# Autodesk Inventor assembly: Full_Field_V5.3_Full_Detail
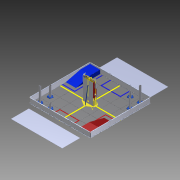
[picture p0: Inventor's stored thumbnail of the model, 180x180]
Saved by Autodesk Inventor 2015 (Build 190159000, 159)
## iProperties
Created: 2015-04-21
Part Number: Full_Field_V5.3_Full_Detail
Document SubType Name: Assembly
Designer: David Tenney
Author: David Tenney
Title: LR15 Full Field V5.3 Full Detail.STEP
Description: STEP AP214
Creation Date: 2014-09-08
Sending System: SolidWorks 2014
Preprocessor: SwSTEP 2.0
## Documents named in this file (10)
- C:\Users\David Tenney\Documents\GitHub\CAD\Field\Imported Components\Full_Field_V5.3_Full_Detail\Full_Field_V5.3_Full_Detail.iam
- C:\Users\David Tenney\Documents\GitHub\CAD\Field\Imported Components\Full_Field_V5.3_Full_Detail\Center Tower 4.4r.iam
- C:\Users\David Tenney\Documents\GitHub\CAD\Field\Imported Components\Full_Field_V5.3_Full_Detail\Bucket ramp v4.iam
- C:\Users\David Tenney\Documents\GitHub\CAD\Field\Imported Components\Full_Field_V5.3_Full_Detail\Player Station.ipt
- C:\Users\David Tenney\Documents\GitHub\CAD\Field\Imported Components\Full_Field_V5.3_Full_Detail\Final Rev1 - Pentagon Goal - 30cm.iam
- C:\Users\David Tenney\Documents\GitHub\CAD\Field\Imported Components\Full_Field_V5.3_Full_Detail\Final Rev1 - Pentagon Goal - 90cm.iam
- C:\Users\David Tenney\Documents\GitHub\CAD\Field\Imported Components\Full_Field_V5.3_Full_Detail\Final Rev1 - Pentagon Goal - 60cm.iam
- C:\Users\David Tenney\Documents\GitHub\CAD\Field\Imported Components\Full_Field_V5.3_Full_Detail\FTC Field Asm.iam
- C:\Users\David Tenney\Documents\GitHub\CAD\Field\Tile Field.iam
- C:\Users\David Tenney\Documents\GitHub\CAD\Field\Bucket ramp v4 Blue.iam
## Components (13 placed, 13 different names)
1. Tile Field_1 [sub-assembly] — Mate:5, Mate:6, Mate:7, Mate:8, Mate:9, Mate:10
2. Center Tower 4.4r_2 [sub-assembly] — Mate:10, Angle:1, Mate:11
3. Bucket ramp v4_3 [sub-assembly] — Mate:3, Mate:4, Mate:6
4. Bucket ramp v4_4 [sub-assembly] — Mate:1, Mate:2, Mate:5
5. Player Station_5
6. Player Station_6
7. Final Rev1 - Pentagon Goal - 30cm_7 [sub-assembly]
8. Final Rev1 - Pentagon Goal - 90cm_8 [sub-assembly]
9. Final Rev1 - Pentagon Goal - 60cm_9 [sub-assembly]
10. Final Rev1 - Pentagon Goal - 30cm_10 [sub-assembly]
11. Final Rev1 - Pentagon Goal - 90cm_11 [sub-assembly]
12. Final Rev1 - Pentagon Goal - 60cm_12 [sub-assembly]
13. FTC Field Asm_13 [sub-assembly] — Mate:1, Mate:2, Mate:3, Mate:4, Mate:7, Mate:8, Mate:9, Angle:1, Mate:11
## Relationships (12: Mate 11, Angle 1)
- Mate:1: Bucket ramp v4_4 ↔ FTC Field Asm_13
- Mate:2: Bucket ramp v4_4 ↔ FTC Field Asm_13
- Mate:3: Bucket ramp v4_3 ↔ FTC Field Asm_13
- Mate:4: Bucket ramp v4_3 ↔ FTC Field Asm_13
- Mate:5: Tile Field_1 ↔ Bucket ramp v4_4
- Mate:6: Tile Field_1 ↔ Bucket ramp v4_3
- Mate:7: Tile Field_1 ↔ FTC Field Asm_13
- Mate:8: Tile Field_1 ↔ FTC Field Asm_13
- Mate:9: Tile Field_1 ↔ FTC Field Asm_13
- Mate:10: Tile Field_1 ↔ Center Tower 4.4r_2
- Angle:1 (0 deg): Center Tower 4.4r_2 ↔ FTC Field Asm_13
- Mate:11: Center Tower 4.4r_2 ↔ FTC Field Asm_13
